# Autodesk Inventor assembly: PCB2_0
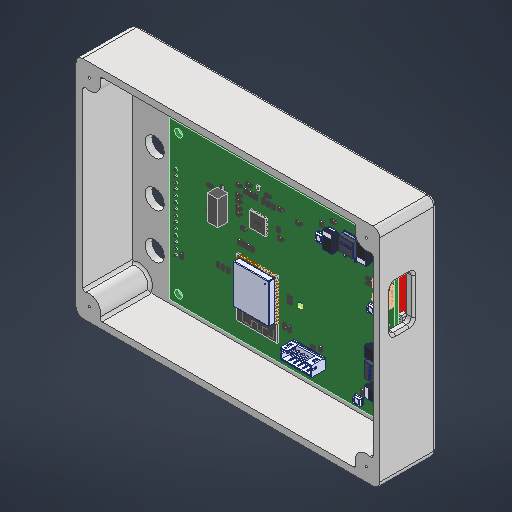
[picture p0: Inventor's stored thumbnail of the model, 512x512]
Saved by Autodesk Inventor 2026.2 (Build 302298000, 298)
## iProperties
Company: Open CASCADE
Created: 2026-01-11
Part Number: PCB2_0
Description: Open CASCADE Model
Document SubType Name: Assembly
Designer: Wellytom
Authority: Unknown
Title: Open CASCADE Shape Model
Author: Author
Sending System: Open CASCADE 7.5
Preprocessor: Open CASCADE STEP processor 7.5
## Documents named in this file (64)
- C:\Users\Wellytom\Documents\GitHub\TCC\altium\TCC01_v2\PCB2_0\PCB2_0\PCB2_0.iam
- C:\Users\Wellytom\Documents\GitHub\TCC\altium\TCC01_v2\PCB2_0\PCB2_0\Board.iam
- C:\Users\Wellytom\Documents\GitHub\TCC\altium\TCC01_v2\PCB2_0\PCB2_0\D4.iam
- C:\Users\Wellytom\Documents\GitHub\TCC\altium\TCC01_v2\PCB2_0\PCB2_0\R26.iam
- C:\Users\Wellytom\Documents\GitHub\TCC\altium\TCC01_v2\PCB2_0\PCB2_0\R25.iam
- C:\Users\Wellytom\Documents\GitHub\TCC\altium\TCC01_v2\PCB2_0\PCB2_0\R24.iam
- C:\Users\Wellytom\Documents\GitHub\TCC\altium\TCC01_v2\PCB2_0\PCB2_0\R20.iam
- C:\Users\Wellytom\Documents\GitHub\TCC\altium\TCC01_v2\PCB2_0\PCB2_0\R19.iam
- C:\Users\Wellytom\Documents\GitHub\TCC\altium\TCC01_v2\PCB2_0\PCB2_0\R18.iam
- C:\Users\Wellytom\Documents\GitHub\TCC\altium\TCC01_v2\PCB2_0\PCB2_0\R17.iam
- C:\Users\Wellytom\Documents\GitHub\TCC\altium\TCC01_v2\PCB2_0\PCB2_0\R16.iam
- C:\Users\Wellytom\Documents\GitHub\TCC\altium\TCC01_v2\PCB2_0\PCB2_0\R15.iam
- C:\Users\Wellytom\Documents\GitHub\TCC\altium\TCC01_v2\PCB2_0\PCB2_0\Y1.iam
- C:\Users\Wellytom\Documents\GitHub\TCC\altium\TCC01_v2\PCB2_0\PCB2_0\U4.iam
- C:\Users\Wellytom\Documents\GitHub\TCC\altium\TCC01_v2\PCB2_0\PCB2_0\U3.iam
- C:\Users\Wellytom\Documents\GitHub\TCC\altium\TCC01_v2\PCB2_0\PCB2_0\U2.iam
- C:\Users\Wellytom\Documents\GitHub\TCC\altium\TCC01_v2\PCB2_0\PCB2_0\U1.iam
- C:\Users\Wellytom\Documents\GitHub\TCC\altium\TCC01_v2\PCB2_0\PCB2_0\R14.iam
- C:\Users\Wellytom\Documents\GitHub\TCC\altium\TCC01_v2\PCB2_0\PCB2_0\R13.iam
- C:\Users\Wellytom\Documents\GitHub\TCC\altium\TCC01_v2\PCB2_0\PCB2_0\R12.iam
- C:\Users\Wellytom\Documents\GitHub\TCC\altium\TCC01_v2\PCB2_0\PCB2_0\R11.iam
- C:\Users\Wellytom\Documents\GitHub\TCC\altium\TCC01_v2\PCB2_0\PCB2_0\R10.iam
- C:\Users\Wellytom\Documents\GitHub\TCC\altium\TCC01_v2\PCB2_0\PCB2_0\R9.iam
- C:\Users\Wellytom\Documents\GitHub\TCC\altium\TCC01_v2\PCB2_0\PCB2_0\R8.iam
- C:\Users\Wellytom\Documents\GitHub\TCC\altium\TCC01_v2\PCB2_0\PCB2_0\R5.iam
- C:\Users\Wellytom\Documents\GitHub\TCC\altium\TCC01_v2\PCB2_0\PCB2_0\R4.iam
- C:\Users\Wellytom\Documents\GitHub\TCC\altium\TCC01_v2\PCB2_0\PCB2_0\R3.iam
- C:\Users\Wellytom\Documents\GitHub\TCC\altium\TCC01_v2\PCB2_0\PCB2_0\R2.iam
- C:\Users\Wellytom\Documents\GitHub\TCC\altium\TCC01_v2\PCB2_0\PCB2_0\R1.iam
- C:\Users\Wellytom\Documents\GitHub\TCC\altium\TCC01_v2\PCB2_0\PCB2_0\LD3.iam
- C:\Users\Wellytom\Documents\GitHub\TCC\altium\TCC01_v2\PCB2_0\PCB2_0\LD2.iam
- C:\Users\Wellytom\Documents\GitHub\TCC\altium\TCC01_v2\PCB2_0\PCB2_0\LD1.iam
- C:\Users\Wellytom\Documents\GitHub\TCC\altium\TCC01_v2\PCB2_0\PCB2_0\LCD1.iam
- C:\Users\Wellytom\Documents\GitHub\TCC\altium\TCC01_v2\PCB2_0\PCB2_0\J1.iam
- C:\Users\Wellytom\Documents\GitHub\TCC\altium\TCC01_v2\PCB2_0\PCB2_0\D1.iam
- C:\Users\Wellytom\Documents\GitHub\TCC\altium\TCC01_v2\PCB2_0\PCB2_0\CN1.iam
- C:\Users\Wellytom\Documents\GitHub\TCC\altium\TCC01_v2\PCB2_0\PCB2_0\C28.iam
- C:\Users\Wellytom\Documents\GitHub\TCC\altium\TCC01_v2\PCB2_0\PCB2_0\C27.iam
- C:\Users\Wellytom\Documents\GitHub\TCC\altium\TCC01_v2\PCB2_0\PCB2_0\C26.iam
- C:\Users\Wellytom\Documents\GitHub\TCC\altium\TCC01_v2\PCB2_0\PCB2_0\C25.iam
- C:\Users\Wellytom\Documents\GitHub\TCC\altium\TCC01_v2\PCB2_0\PCB2_0\C24.iam
- C:\Users\Wellytom\Documents\GitHub\TCC\altium\TCC01_v2\PCB2_0\PCB2_0\C23.iam
- C:\Users\Wellytom\Documents\GitHub\TCC\altium\TCC01_v2\PCB2_0\PCB2_0\C22.iam
- C:\Users\Wellytom\Documents\GitHub\TCC\altium\TCC01_v2\PCB2_0\PCB2_0\C21.iam
- C:\Users\Wellytom\Documents\GitHub\TCC\altium\TCC01_v2\PCB2_0\PCB2_0\C20.iam
- C:\Users\Wellytom\Documents\GitHub\TCC\altium\TCC01_v2\PCB2_0\PCB2_0\C19.iam
- C:\Users\Wellytom\Documents\GitHub\TCC\altium\TCC01_v2\PCB2_0\PCB2_0\C18.iam
- C:\Users\Wellytom\Documents\GitHub\TCC\altium\TCC01_v2\PCB2_0\PCB2_0\C17.iam
- C:\Users\Wellytom\Documents\GitHub\TCC\altium\TCC01_v2\PCB2_0\PCB2_0\C16.iam
- C:\Users\Wellytom\Documents\GitHub\TCC\altium\TCC01_v2\PCB2_0\PCB2_0\C15.iam
- C:\Users\Wellytom\Documents\GitHub\TCC\altium\TCC01_v2\PCB2_0\PCB2_0\C14.iam
- C:\Users\Wellytom\Documents\GitHub\TCC\altium\TCC01_v2\PCB2_0\PCB2_0\C13.iam
- C:\Users\Wellytom\Documents\GitHub\TCC\altium\TCC01_v2\PCB2_0\PCB2_0\C11.iam
- C:\Users\Wellytom\Documents\GitHub\TCC\altium\TCC01_v2\PCB2_0\PCB2_0\C10.iam
- C:\Users\Wellytom\Documents\GitHub\TCC\altium\TCC01_v2\PCB2_0\PCB2_0\C9.iam
- C:\Users\Wellytom\Documents\GitHub\TCC\altium\TCC01_v2\PCB2_0\PCB2_0\C8.iam
- C:\Users\Wellytom\Documents\GitHub\TCC\altium\TCC01_v2\PCB2_0\PCB2_0\C7.iam
- C:\Users\Wellytom\Documents\GitHub\TCC\altium\TCC01_v2\PCB2_0\PCB2_0\C6.iam
- C:\Users\Wellytom\Documents\GitHub\TCC\altium\TCC01_v2\PCB2_0\PCB2_0\C5.iam
- C:\Users\Wellytom\Documents\GitHub\TCC\altium\TCC01_v2\PCB2_0\PCB2_0\C4.iam
- C:\Users\Wellytom\Documents\GitHub\TCC\altium\TCC01_v2\PCB2_0\PCB2_0\C3.iam
- C:\Users\Wellytom\Documents\GitHub\TCC\altium\TCC01_v2\PCB2_0\PCB2_0\C2.iam
- C:\Users\Wellytom\Documents\GitHub\TCC\altium\TCC01_v2\PCB2_0\PCB2_0\C1.iam
- C:\Users\Wellytom\Documents\GitHub\TCC\inventor\wash\GabineteWash2.ipt
## Components (63 placed, 63 different names)
1. Board_2 [sub-assembly]
2. D4_15 [sub-assembly]
3. R26_17 [sub-assembly]
4. R25_19 [sub-assembly]
5. R24_21 [sub-assembly]
6. R20_23 [sub-assembly]
7. R19_25 [sub-assembly]
8. R18_27 [sub-assembly]
9. R17_29 [sub-assembly]
10. R16_31 [sub-assembly]
11. R15_33 [sub-assembly]
12. Y1_37 [sub-assembly]
13. U4_39 [sub-assembly]
14. U3_41 [sub-assembly]
15. U2_43 [sub-assembly]
16. U1_49 [sub-assembly]
17. R14_51 [sub-assembly]
18. R13_53 [sub-assembly]
19. R12_55 [sub-assembly]
20. R11_57 [sub-assembly]
21. R10_59 [sub-assembly]
22. R9_61 [sub-assembly]
23. R8_63 [sub-assembly]
24. R5_65 [sub-assembly]
25. R4_67 [sub-assembly]
26. R3_69 [sub-assembly]
27. R2_71 [sub-assembly]
28. R1_73 [sub-assembly]
29. LD3_75 [sub-assembly]
30. LD2_77 [sub-assembly]
31. LD1_79 [sub-assembly]
32. LCD1_81 [sub-assembly] — Flush:1, Flush:2
33. J1_83 [sub-assembly]
34. D1_88 [sub-assembly]
35. CN1_90 [sub-assembly]
36. C28_92 [sub-assembly]
37. C27_94 [sub-assembly]
38. C26_96 [sub-assembly]
39. C25_98 [sub-assembly]
40. C24_100 [sub-assembly]
41. C23_102 [sub-assembly]
42. C22_104 [sub-assembly]
43. C21_106 [sub-assembly]
44. C20_108 [sub-assembly]
45. C19_110 [sub-assembly]
46. C18_112 [sub-assembly]
47. C17_114 [sub-assembly]
48. C16_116 [sub-assembly]
49. C15_118 [sub-assembly]
50. C14_120 [sub-assembly]
51. C13_122 [sub-assembly]
52. C11_124 [sub-assembly]
53. C10_126 [sub-assembly]
54. C9_128 [sub-assembly]
55. C8_130 [sub-assembly]
56. C7_132 [sub-assembly]
57. C6_134 [sub-assembly]
58. C5_136 [sub-assembly]
59. C4_138 [sub-assembly]
60. C3_140 [sub-assembly]
61. C2_142 [sub-assembly]
62. C1_144 [sub-assembly]
63. GabineteWash2:1 — Flush:1, Flush:2
## Relationships (2: Flush 2)
- Flush:1: LCD1_81 ↔ GabineteWash2:1
- Flush:2: LCD1_81 ↔ GabineteWash2:1
